# Autodesk Inventor assembly: LeftBottomTube
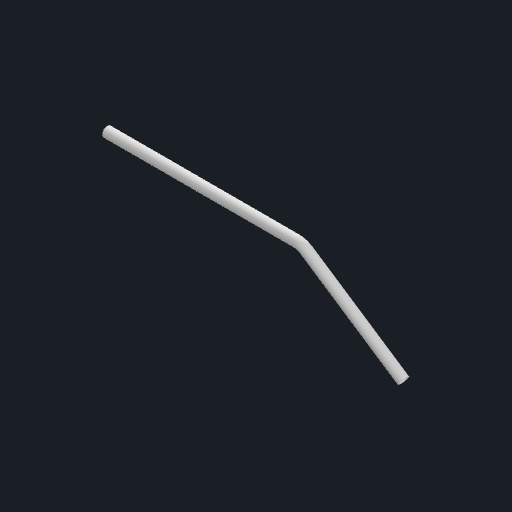
[picture p0: Inventor's stored thumbnail of the model, 512x512]
Saved by Autodesk Inventor 2025.2 (Build 292293000, 293)
## iProperties
Created: 2025-04-01
Part Number: LeftBottomTube
Document SubType Name: Assembly
Designer: valer
Author: valer
## Documents named in this file (2)
- C:\Users\valer\Desktop\str1ker\cad\LeftBottomTube.iam
- C:\Users\valer\Desktop\str1ker\cad\ChestLeftBottomTube.ipt
## Components (1 placed, 1 different names)
1. ChestLeftBottomTube:1 — Mate:1, Mate:2
## Relationships (2: Mate 2)
- Mate:1: ChestLeftBottomTube:1
- Mate:2: ChestLeftBottomTube:1
